# Autodesk Inventor assembly: Assembly3
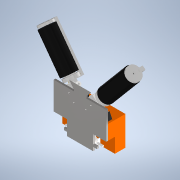
[picture p0: Inventor's stored thumbnail of the model, 180x180]
Saved by Autodesk Inventor 2022.3 (Build 263350000, 350)
## iProperties
Created: 2022-11-17
Part Number: Assembly3
Document SubType Name: Assembly
Designer: komputer
Author: komputer
## Documents named in this file (6)
- C:\Users\komputer\Desktop\Krab\Assembly3.iam
- C:\Users\komputer\Part12.ipt
- C:\Users\komputer\pałka.iam
- C:\Users\komputer\Desktop\Projekty\ILYT_MS\n20 motor.ipt
- C:\Users\komputer\Part16.ipt
- C:\Users\komputer\Part17.ipt
## Components (7 placed, 5 different names)
1. Part12:1 — Mate:1, Mate:2, Mate:3, Mate:4, Flush:1, Mate:5, Flush:2, Mate:6, Flush:3, Flush:4
2. pałka:1 [sub-assembly] — Mate:1, Mate:2
3. pałka:2 [sub-assembly] — Mate:3, Mate:4
4. n20 motor:1 — Flush:2, Mate:6
5. n20 motor:2 — Flush:1, Mate:5
6. Part16:1 — Flush:3
7. Part17:1 — Flush:4
## Relationships (10: Mate 6, Flush 4)
- Mate:1: Part12:1 ↔ pałka:1
- Mate:2: Part12:1 ↔ pałka:1
- Mate:3: Part12:1 ↔ pałka:2
- Mate:4: Part12:1 ↔ pałka:2
- Flush:1: Part12:1 ↔ n20 motor:2
- Mate:5: Part12:1 ↔ n20 motor:2
- Flush:2: Part12:1 ↔ n20 motor:1
- Mate:6: Part12:1 ↔ n20 motor:1
- Flush:3: Part12:1 ↔ Part16:1
- Flush:4: Part12:1 ↔ Part17:1
